# Autodesk Inventor assembly: Front Panel Assembly
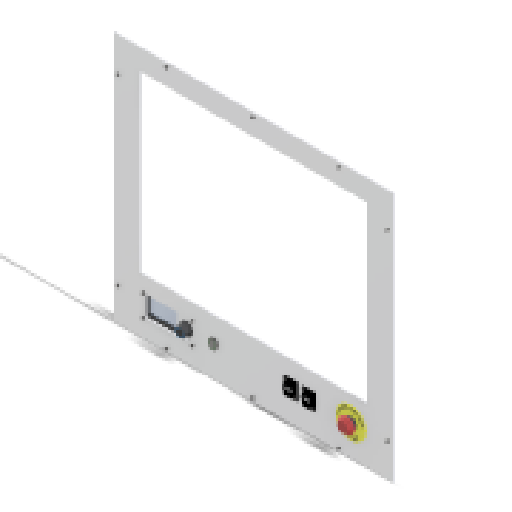
[picture p0: Inventor's stored thumbnail of the model, 512x512]
Saved by Autodesk Inventor 2023.2 (Build 272271000, 271)
## iProperties
Created: 2023-02-06
Part Number: Front Panel Assembly
Document SubType Name: Assembly
Designer: remop
Author: remop
## Documents named in this file (11)
- C:\Users\remop\OneDrive\Documents\Inventor\3D Printers\LuEVO\Mk5_FullKinematic\Frame and Panels\Front Panel Assembly.iam
- C:\Users\remop\OneDrive\Documents\Inventor\3D Printers\LuEVO\Mk5_FullKinematic\Frame and Panels\Front Panel.ipt
- C:\Users\remop\OneDrive\Documents\Inventor\Content Center Files\R2023\en-US\AS 1420\AS 1420 - 1973 - M3 x 6.ipt
- C:\Users\remop\OneDrive\Documents\Inventor\3D Printers\LuEVO\Mk5_FullKinematic\Electronics\Baseframe Electronics\E-Stop Plate (Yellow).ipt
- C:\Users\remop\OneDrive\Documents\Inventor\3D Printers\LuEVO\Mk5_FullKinematic\Electronics\Baseframe Electronics\E-Stop Plate (Black).ipt
- C:\Users\remop\OneDrive\Documents\Inventor\3D Printers\LuEVO\Mk5_FullKinematic\Electronics\Baseframe Electronics\E-Stop Dummy.ipt
- C:\Users\remop\OneDrive\Documents\Inventor\3D Printers\LuEVO\Mk5_FullKinematic\Electronics\BTT Mini 12864 V1.0.ipt
- C:\Users\remop\OneDrive\Documents\Inventor\3D Printers\LuEVO\Mk5_FullKinematic\Electronics\Delock Panel Connector.ipt
- C:\Users\remop\OneDrive\Documents\Inventor\3D Printers\LuEVO\Mk5_FullKinematic\Electronics\Power Button.ipt
- C:\Users\remop\OneDrive\Documents\Inventor\Content Center Files\R2023\en-US\AS 1420\AS 1420 - 1973 - M3 x 16.ipt
- C:\Users\remop\OneDrive\Documents\Inventor\Content Center Files\R2023\en-US\AS 1420\AS 1420 - 1973 - M3 x 12.ipt
## Components (26 placed, 10 different names)
1. Front Panel:1 — Insert:1, Insert:2, Insert:3, Insert:4, Insert:5, Insert:6, Insert:7, Insert:8, Insert:9, Insert:10, Rotational:1, Flush:1, Flush:2, Flush:3, Rigid:3, Rotational:2, Insert:11, Insert:12, Insert:13, Insert:14
2. AS 1420 - Metric M3 x 6:1 — Insert:1
3. AS 1420 - Metric M3 x 6:2 — Insert:2
4. AS 1420 - Metric M3 x 6:3 — Insert:3
5. AS 1420 - Metric M3 x 6:4 — Insert:4
6. AS 1420 - Metric M3 x 6:5 — Insert:5
7. AS 1420 - Metric M3 x 6:6 — Insert:6
8. AS 1420 - Metric M3 x 6:7 — Insert:7
9. AS 1420 - Metric M3 x 6:8 — Insert:8
10. AS 1420 - Metric M3 x 6:9 — Insert:9
11. AS 1420 - Metric M3 x 6:10 — Insert:10
12. E-Stop Plate (Yellow):1 — Rotational:1
13. E-Stop Plate (Black):1
14. E-Stop Dummy:1
15. BTT Mini 12864 V1.0:1 — Flush:1, Flush:2, Flush:3
16. Delock Panel Connector:1 — Rigid:3, Insert:15, Insert:16
17. Delock Panel Connector:2 — Rotational:2, Mate:1, Mate:2, Mate:3, Mate:4
18. Power Button:1
19. AS 1420 - Metric M3 x 16:1 — Insert:11
20. AS 1420 - Metric M3 x 16:2 — Insert:12
21. AS 1420 - Metric M3 x 16:3 — Insert:13
22. AS 1420 - Metric M3 x 16:4 — Insert:14
23. AS 1420 - Metric M3 x 12:1 — Insert:15
24. AS 1420 - Metric M3 x 12:2 — Insert:16
25. AS 1420 - Metric M3 x 12:3 — Mate:1, Mate:2
26. AS 1420 - Metric M3 x 12:4 — Mate:3, Mate:4
## Relationships (26: Insert 16, Mate 4, Flush 3, RevoluteJoint 2, WeldJoint 1)
- Insert:1: Front Panel:1 ↔ AS 1420 - Metric M3 x 6:1
- Insert:2: Front Panel:1 ↔ AS 1420 - Metric M3 x 6:2
- Insert:3: Front Panel:1 ↔ AS 1420 - Metric M3 x 6:3
- Insert:4: Front Panel:1 ↔ AS 1420 - Metric M3 x 6:4
- Insert:5: Front Panel:1 ↔ AS 1420 - Metric M3 x 6:5
- Insert:6: Front Panel:1 ↔ AS 1420 - Metric M3 x 6:6
- Insert:7: Front Panel:1 ↔ AS 1420 - Metric M3 x 6:7
- Insert:8: Front Panel:1 ↔ AS 1420 - Metric M3 x 6:8
- Insert:9: Front Panel:1 ↔ AS 1420 - Metric M3 x 6:9
- Insert:10: Front Panel:1 ↔ AS 1420 - Metric M3 x 6:10
- Rotational:1 [RevoluteJoint]: Front Panel:1 ↔ E-Stop Plate (Yellow):1
- Flush:1 (3 mm): Front Panel:1 ↔ BTT Mini 12864 V1.0:1
- Flush:2 (27 mm): Front Panel:1 ↔ BTT Mini 12864 V1.0:1
- Flush:3 (380 mm): Front Panel:1 ↔ BTT Mini 12864 V1.0:1
- Rigid:3 [WeldJoint]: Front Panel:1 ↔ Delock Panel Connector:1
- Rotational:2 [RevoluteJoint]: Front Panel:1 ↔ Delock Panel Connector:2
- Insert:11: Front Panel:1 ↔ AS 1420 - Metric M3 x 16:1
- Insert:12: Front Panel:1 ↔ AS 1420 - Metric M3 x 16:2
- Insert:13: Front Panel:1 ↔ AS 1420 - Metric M3 x 16:3
- Insert:14: Front Panel:1 ↔ AS 1420 - Metric M3 x 16:4
- Insert:15: Delock Panel Connector:1 ↔ AS 1420 - Metric M3 x 12:1
- Insert:16: Delock Panel Connector:1 ↔ AS 1420 - Metric M3 x 12:2
- Mate:1: Delock Panel Connector:2 ↔ AS 1420 - Metric M3 x 12:3
- Mate:2: Delock Panel Connector:2 ↔ AS 1420 - Metric M3 x 12:3
- Mate:3: Delock Panel Connector:2 ↔ AS 1420 - Metric M3 x 12:4
- Mate:4: Delock Panel Connector:2 ↔ AS 1420 - Metric M3 x 12:4
